# Autodesk Inventor assembly: Übertragung des Zahnriemens
Saved by Autodesk Inventor 2016 (Build 200138000, 138)
## iProperties
Created: 2015-08-24
Part Number: Übertragung des Zahnriemens
Document SubType Name: Assembly
Designer: 4ndreas
Mass: 16.2956 g
Surface Area: 94.7866 cm^2
Volume: 6.65808 cm^3
Density: 2.44749 g/cm^3
ClientObjectVersion: 1
Author: 4ndreas
## Documents named in this file (3)
- C:\Users\4ndreas\Documents\Inventor\RobotARM v2\v4\Ellbow\Konstruktions-Assistent\Übertragung des Zahnriemens2.iam
- C:\Users\4ndreas\Documents\Inventor\RobotARM v2\v4\Ellbow\Konstruktions-Assistent\Zahnriemen2.ipt
- C:\Users\4ndreas\Documents\Inventor\RobotARM v2\v4\Ellbow\Konstruktions-Assistent\Flache Riemenscheibe12.ipt
## Components (2 placed, 2 different names)
1. Zahnriemen:1 — Fluchtend:1, Passend:1
2. Flache Riemenscheibe1:1 — Fluchtend:1, Passend:1
## Relationships (2: Flush 1, Mate 1)
- Fluchtend:1 [Flush]: Zahnriemen:1 ↔ Flache Riemenscheibe1:1
- Passend:1 [Mate]: Zahnriemen:1 ↔ Flache Riemenscheibe1:1
